# Autodesk Inventor assembly: A2017_T4_14
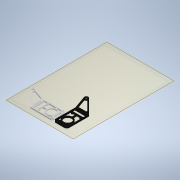
[picture p0: Inventor's stored thumbnail of the model, 180x180]
Saved by Autodesk Inventor 2020 (Build 240168000, 168)
## iProperties
Created: 2021-08-27
Part Number: A2017_T4_14
Document SubType Name: Assembly
Designer: Masato
Author: Masato
## Documents named in this file (4)
- D:\GitHub\inventor\SUSTAINA-OP\Cam\A2017_T4_14.iam
- D:\GitHub\inventor\SUSTAINA-OP\Cam\DisposableBoard.ipt
- D:\GitHub\inventor\SUSTAINA-OP\UpperBody\Trunk\Trunk_shoulder_frame.ipt
- D:\GitHub\inventor\SUSTAINA-OP\UpperBody\Trunk\Trunk_shoulder_frame_MIR.ipt
## Components (3 placed, 3 different names)
1. DisposableBoard:1 — メイト:2, メイト:1, フラッシュ:1, フラッシュ:2, メイト:6, メイト:13, メイト:14, メイト:15, 正接:1
2. Trunk_shoulder_frame_MIR:1 — メイト:6, メイト:13, メイト:16, 正接:1
3. Trunk_shoulder_frame:1 — メイト:14, メイト:15, メイト:16
## Relationships (10: Mate 7, Flush 2, Tangent 1)
- メイト:2 [Mate]: DisposableBoard:1
- メイト:1 [Mate]: DisposableBoard:1
- フラッシュ:1 [Flush]: DisposableBoard:1
- フラッシュ:2 [Flush]: DisposableBoard:1
- メイト:6 [Mate]: DisposableBoard:1 ↔ Trunk_shoulder_frame_MIR:1
- メイト:13 [Mate] (2 mm): DisposableBoard:1 ↔ Trunk_shoulder_frame_MIR:1
- メイト:14 [Mate]: DisposableBoard:1 ↔ Trunk_shoulder_frame:1
- メイト:15 [Mate] (2 mm): DisposableBoard:1 ↔ Trunk_shoulder_frame:1
- メイト:16 [Mate] (2.5 mm): Trunk_shoulder_frame_MIR:1 ↔ Trunk_shoulder_frame:1
- 正接:1 [Tangent] (2 mm): DisposableBoard:1 ↔ Trunk_shoulder_frame_MIR:1
